# Autodesk Inventor assembly: 48-0070
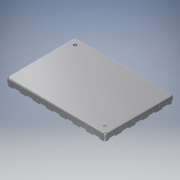
[picture p0: Inventor's stored thumbnail of the model, 180x180]
Saved by Autodesk Inventor 2018 (Build 220112000, 112)
## iProperties
Created: 2019-09-25
Part Number: 48-0070
Document SubType Name: Assembly
Designer: Bradley
Author: Bradley
## Documents named in this file (3)
- C:\Users\Bradley\Documents\GitHub\Resources\SupplierDocuments\48 - Hardware\48-0070\48-0070.iam
- C:\Users\Bradley\Documents\GitHub\Resources\SupplierDocuments\48 - Hardware\48-0070\48-0070.ipt
- C:\Users\Bradley\Documents\GitHub\Resources\SupplierDocuments\48 - Hardware\48-0071\48-0071.ipt
## Components (2 placed, 2 different names)
1. 48-0070:1 — Flush:1, Flush:2, Mate:1
2. 48-0071:1 — Flush:1, Flush:2, Mate:1
## Relationships (3: Flush 2, Mate 1)
- Flush:1: 48-0070:1 ↔ 48-0071:1
- Flush:2: 48-0070:1 ↔ 48-0071:1
- Mate:1: 48-0070:1 ↔ 48-0071:1
